# Autodesk Inventor assembly: Assembly Mount Assembly
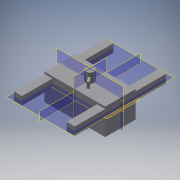
[picture p0: Inventor's stored thumbnail of the model, 180x180]
Saved by Autodesk Inventor 2019 (Build 230136000, 136)
## iProperties
Created: 2021-05-09
Part Number: Assembly Mount Assembly
Document SubType Name: Assembly
Designer: Eric
Author: Eric
## Documents named in this file (3)
- C:\Users\Eric\Documents\! - Uni\Year 4\MENG-Robot-Fab-Project\Models\For_Optimiser\Assembly Mount Assembly\Assembly Mount Assembly.iam
- C:\Users\Eric\Documents\! - Uni\Year 4\MENG-Robot-Fab-Project\Models\For_Optimiser\Assembly Mount Assembly\Assembly Mount Base.ipt
- C:\Users\Eric\Documents\! - Uni\Year 4\MENG-Robot-Fab-Project\Models\For_Optimiser\Assembly Mount Assembly\Assembly Mount Rack.ipt
## Components (2 placed, 2 different names)
1. Assembly Mount Base:1 — Mate:1, Mate:2, Flush:1
2. Assembly Mount Rack:1 — Mate:1, Mate:2, Flush:1
## Relationships (3: Mate 2, Flush 1)
- Mate:1: Assembly Mount Base:1 ↔ Assembly Mount Rack:1
- Mate:2 (11.5 mm): Assembly Mount Base:1 ↔ Assembly Mount Rack:1
- Flush:1: Assembly Mount Base:1 ↔ Assembly Mount Rack:1
